# Autodesk Inventor assembly: Tire
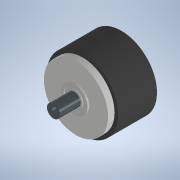
[picture p0: Inventor's stored thumbnail of the model, 180x180]
Saved by Autodesk Inventor 2022 (Build 260153000, 153)
## iProperties
Created: 2021-09-23
Part Number: Tire
Document SubType Name: Assembly
Designer: shiok
Mass: 6.37362 g
Surface Area: 59.289 cm^2
Volume: 3.61915 cm^3
Density: 1.76108 g/cm^3
Author: shiok
## Documents named in this file (7)
- C:\Users\Yazawa\Documents\GitHub\murakumo\inventor\Tire.iam
- C:\Users\Yazawa\Documents\GitHub\murakumo\inventor\Tire.ipt
- C:\Users\Yazawa\Documents\GitHub\murakumo\inventor\shaft.ipt
- C:\Users\Yazawa\Documents\GitHub\murakumo\inventor\wheelcap.ipt
- C:\Users\Yazawa\Documents\GitHub\murakumo\inventor\wheel_v2.ipt
- C:\Users\Yazawa\Documents\GitHub\murakumo\inventor\FL674ZZ.ipt
- C:\Users\Yazawa\Documents\GitHub\murakumo\inventor\Tire\デザイン アクセラレータ\平歯車2.iam
## Components (7 placed, 6 different names)
1. Tire:1 — メイト:1, フラッシュ:1
2. shaft:1 — メイト:8, フラッシュ:2
3. wheelcap:1 — メイト:4, メイト:5, メイト:6, メイト:7
4. wheel_v2:1 — メイト:1, フラッシュ:1, メイト:2, メイト:3, メイト:6, メイト:7
5. FL674ZZ:1 — メイト:2, メイト:3, メイト:8
6. FL674ZZ:2 — メイト:4, メイト:5, フラッシュ:2
7. 平歯車:1 [sub-assembly]
## Relationships (10: Mate 8, Flush 2)
- メイト:1 [Mate]: Tire:1 ↔ wheel_v2:1
- フラッシュ:1 [Flush]: Tire:1 ↔ wheel_v2:1
- メイト:2 [Mate]: wheel_v2:1 ↔ FL674ZZ:1
- メイト:3 [Mate]: wheel_v2:1 ↔ FL674ZZ:1
- メイト:4 [Mate]: wheelcap:1 ↔ FL674ZZ:2
- メイト:5 [Mate]: wheelcap:1 ↔ FL674ZZ:2
- メイト:6 [Mate]: wheelcap:1 ↔ wheel_v2:1
- メイト:7 [Mate]: wheelcap:1 ↔ wheel_v2:1
- メイト:8 [Mate]: shaft:1 ↔ FL674ZZ:1
- フラッシュ:2 [Flush]: shaft:1 ↔ FL674ZZ:2
